# Autodesk Inventor assembly: MontagemREV0
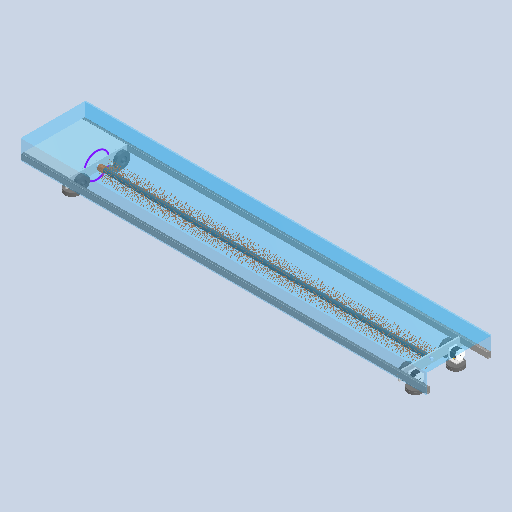
[picture p0: Inventor's stored thumbnail of the model, 512x512]
Saved by Autodesk Inventor 2025.3 (Build 293356030, 356C)
## iProperties
Created: 2025-11-04
Part Number: MontagemREV0
Document SubType Name: Assembly
Designer: Rubens
Author: Rubens
## Documents named in this file (12)
- C:\Users\Rubens\Downloads\Limpador\MontagemREV0.iam
- C:\Users\Rubens\Downloads\Limpador\TCC\aaaaaISO 10799-2 - 40x20x2 - 2600.ipt
- C:\Users\Rubens\Downloads\Limpador\TCC\aaaaaPart2.ipt
- C:\Users\Rubens\Downloads\Limpador\TCC\aaaaa22874-100-g-a.ipt
- C:\Users\Rubens\Downloads\Limpador\TCC\aaaaaSuporte Painel1.ipt
- C:\Users\Rubens\Downloads\Limpador\EscovãoFinal.ipt
- C:\Users\Rubens\Downloads\Limpador\EscovãoMID.ipt
- C:\Users\Rubens\Downloads\Limpador\EscovãoInicial.ipt
- C:\Users\Rubens\Downloads\Limpador\Teste Suporte.ipt
- C:\Users\Rubens\Documents\Inventor\Content Center Files\R2025\pt-BR\AS 1420\AS 1420 - 1973 - M12 x 40.ipt
- C:\Users\Rubens\Downloads\Limpador\Teste Placa.ipt
- C:\Users\Rubens\Downloads\Estrutura Placa - REV00\Solar Mounting Structure\Main_Solar_Structure\Main_Solar_Structure\MPN23-12 - MOTOR DE PASSO NEMA 23.ipt
## Components (29 placed, 11 different names)
1. aaaaaISO 10799-2 - 40x20x2 - 2600:1 — Coincidente:1, Coincidente:3, Alinhado:1, Coincidente:5, Alinhado:3, Coincidente:26, Coincidente:27
2. aaaaaISO 10799-2 - 40x20x2 - 2600:2 — Coincidente:2, Coincidente:4, Alinhado:1, Coincidente:8, Alinhado:2, Coincidente:9, Coincidente:10
3. aaaaaPart2:1 — Coincidente:9, Coincidente:10, Alinhado:3, Coincidente:17, Inserir:3, Inserir:4, Coincidente:20, Coincidente:21
4. aaaaaPart2:2 — Coincidente:1, Coincidente:2, Coincidente:3, Coincidente:4, Coincidente:6, Coincidente:7, Inserir:1, Inserir:2, Coincidente:22, Coincidente:23
5. aaaaa22874-100-g-a:1 — Inserir:1
6. aaaaa22874-100-g-a:2 — Inserir:2
7. aaaaa22874-100-g-a:3 — Inserir:3
8. aaaaa22874-100-g-a:4 — Inserir:4
9. aaaaaSuporte Painel1:1 — Coincidente:5, Coincidente:6, Coincidente:7, Coincidente:8, Alinhado:2
10. EscovãoFinal:1 — Coincidente:16, Coincidente:17
11. EscovãoMID:1 — Coincidente:15, Coincidente:16
12. EscovãoInicial:1 — Coincidente:15
13. aaaaa22874-100-g-a:5 — Inserir:9
14. aaaaa22874-100-g-a:6 — Inserir:10
15. Teste Suporte:3 — Coincidente:20, Inserir:7, Inserir:17, Coincidente:29
16. Teste Suporte:4 — Coincidente:21, Inserir:8, Inserir:16, Coincidente:28
17. aaaaa22874-100-g-a:7 — Inserir:7
18. aaaaa22874-100-g-a:8 — Inserir:8
19. Teste Suporte:5 — Coincidente:22, Inserir:9, Coincidente:25, Inserir:11
20. Teste Suporte:6 — Coincidente:23, Inserir:10, Inserir:12, Inserir:13
21. AS 1420 - Métrica M12 x 40:2 — Coincidente:25
22. AS 1420 - Métrica M12 x 40:3 — Inserir:11
23. AS 1420 - Métrica M12 x 40:5 — Inserir:13
24. AS 1420 - Métrica M12 x 40:6 — Inserir:12
25. AS 1420 - Métrica M12 x 40:7 — Inserir:16
26. AS 1420 - Métrica M12 x 40:9 — Inserir:17
27. Teste Placa:1 — Coincidente:26, Coincidente:27
28. MPN23-12 - MOTOR DE PASSO NEMA 23:2 — Coincidente:29
29. MPN23-12 - MOTOR DE PASSO NEMA 23:3 — Coincidente:28
## Relationships (38: Mate 22, Insert 13, Flush 3)
- Coincidente:1 [Mate]: aaaaaISO 10799-2 - 40x20x2 - 2600:1 ↔ aaaaaPart2:2
- Coincidente:2 [Mate]: aaaaaISO 10799-2 - 40x20x2 - 2600:2 ↔ aaaaaPart2:2
- Coincidente:3 [Mate]: aaaaaISO 10799-2 - 40x20x2 - 2600:1 ↔ aaaaaPart2:2
- Coincidente:4 [Mate]: aaaaaISO 10799-2 - 40x20x2 - 2600:2 ↔ aaaaaPart2:2
- Alinhado:1 [Flush]: aaaaaISO 10799-2 - 40x20x2 - 2600:1 ↔ aaaaaISO 10799-2 - 40x20x2 - 2600:2
- Coincidente:5 [Mate]: aaaaaISO 10799-2 - 40x20x2 - 2600:1 ↔ aaaaaSuporte Painel1:1
- Coincidente:6 [Mate]: aaaaaPart2:2 ↔ aaaaaSuporte Painel1:1
- Coincidente:7 [Mate]: aaaaaPart2:2 ↔ aaaaaSuporte Painel1:1
- Coincidente:8 [Mate]: aaaaaISO 10799-2 - 40x20x2 - 2600:2 ↔ aaaaaSuporte Painel1:1
- Alinhado:2 [Flush]: aaaaaISO 10799-2 - 40x20x2 - 2600:2 ↔ aaaaaSuporte Painel1:1
- Coincidente:9 [Mate]: aaaaaISO 10799-2 - 40x20x2 - 2600:2 ↔ aaaaaPart2:1
- Coincidente:10 [Mate]: aaaaaISO 10799-2 - 40x20x2 - 2600:2 ↔ aaaaaPart2:1
- Alinhado:3 [Flush] (190 mm): aaaaaISO 10799-2 - 40x20x2 - 2600:1 ↔ aaaaaPart2:1
- Coincidente:15 [Mate]: EscovãoMID:1 ↔ EscovãoInicial:1
- Coincidente:16 [Mate]: EscovãoFinal:1 ↔ EscovãoMID:1
- Coincidente:17 [Mate]: aaaaaPart2:1 ↔ EscovãoFinal:1
- Inserir:1: aaaaaPart2:2 ↔ aaaaa22874-100-g-a:1
- Inserir:2: aaaaaPart2:2 ↔ aaaaa22874-100-g-a:2
- Inserir:3: aaaaaPart2:1 ↔ aaaaa22874-100-g-a:3
- Inserir:4: aaaaaPart2:1 ↔ aaaaa22874-100-g-a:4
- Coincidente:20 [Mate]: aaaaaPart2:1 ↔ Teste Suporte:3
- Coincidente:21 [Mate]: aaaaaPart2:1 ↔ Teste Suporte:4
- Inserir:7: Teste Suporte:3 ↔ aaaaa22874-100-g-a:7
- Inserir:8: Teste Suporte:4 ↔ aaaaa22874-100-g-a:8
- Coincidente:22 [Mate]: aaaaaPart2:2 ↔ Teste Suporte:5
- Coincidente:23 [Mate]: aaaaaPart2:2 ↔ Teste Suporte:6
- Inserir:9: aaaaa22874-100-g-a:5 ↔ Teste Suporte:5
- Inserir:10: aaaaa22874-100-g-a:6 ↔ Teste Suporte:6
- Coincidente:25 [Mate]: Teste Suporte:5 ↔ AS 1420 - Métrica M12 x 40:2
- Inserir:11: Teste Suporte:5 ↔ AS 1420 - Métrica M12 x 40:3
- Inserir:12: Teste Suporte:6 ↔ AS 1420 - Métrica M12 x 40:6
- Inserir:13: Teste Suporte:6 ↔ AS 1420 - Métrica M12 x 40:5
- Inserir:16: Teste Suporte:4 ↔ AS 1420 - Métrica M12 x 40:7
- Inserir:17: Teste Suporte:3 ↔ AS 1420 - Métrica M12 x 40:9
- Coincidente:26 [Mate]: aaaaaISO 10799-2 - 40x20x2 - 2600:1 ↔ Teste Placa:1
- Coincidente:27 [Mate]: aaaaaISO 10799-2 - 40x20x2 - 2600:1 ↔ Teste Placa:1
- Coincidente:28 [Mate]: Teste Suporte:4 ↔ MPN23-12 - MOTOR DE PASSO NEMA 23:3
- Coincidente:29 [Mate]: Teste Suporte:3 ↔ MPN23-12 - MOTOR DE PASSO NEMA 23:2
## Named parameters: Finish1_Area = 799.295, Finish2_Area = 2027.67, Finish3_Area = 2027.67
note: some values were not read from the file. Shown as the stored number, unit unknown: "Finish1_Area", "Finish2_Area", "Finish3_Area".
